# Autodesk Inventor assembly: LEG
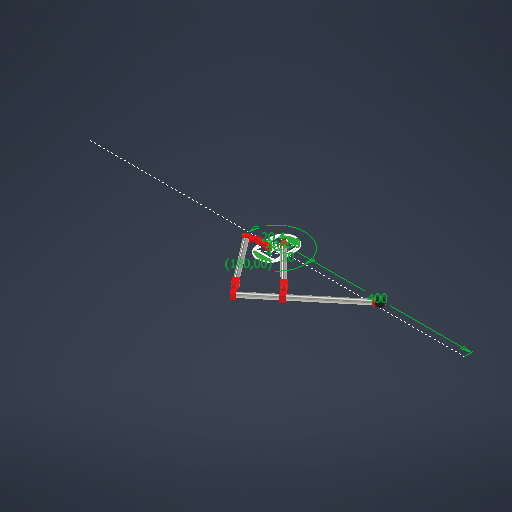
[picture p0: Inventor's stored thumbnail of the model, 512x512]
Saved by Autodesk Inventor 2027 (Build 310192060, 192F)
## iProperties
Created: 2026-08-01
Part Number: LEG
Document SubType Name: Assembly
Designer: User
Author: User
## Documents named in this file (11)
- G:\Github\Hot_dog\Hardware\Leg_concept\LEG.iam
- G:\Github\Hot_dog\Hardware\Leg_concept\Knee.ipt
- G:\Github\Hot_dog\Hardware\Leg_concept\foot.ipt
- G:\Github\Hot_dog\Hardware\Leg_concept\base.ipt
- G:\Github\Hot_dog\Hardware\Leg_concept\tibia.ipt
- G:\Github\Hot_dog\Hardware\Leg_concept\Connector_fill.ipt
- G:\Github\Hot_dog\Hardware\Leg_concept\Connector_hollow.ipt
- G:\Github\Hot_dog\Hardware\Leg_concept\short_tibia.ipt
- G:\Github\Hot_dog\Hardware\Leg_concept\connecting_rod.ipt
- G:\Github\Hot_dog\Hardware\Leg_concept\long_tibia.ipt
- G:\Github\Hot_dog\Hardware\Leg_concept\connector.ipt
## Components (14 placed, 10 different names)
1. Connector_fill:1 — Obrotowe:13, Obrotowe:29
2. Connector_hollow:1 — Obrotowe:23, Obrotowe:28
3. base:1 — Obrotowe:24, Obrotowe:25
4. Connector_hollow:2 — Obrotowe:15
5. tibia:2 — Obrotowe:26
6. connecting_rod:1 — Obrotowe:19, Obrotowe:24
7. connecting_rod:2 — Obrotowe:13, Obrotowe:25
8. Knee:1 — Obrotowe:21, Obrotowe:23
9. foot:1 — Obrotowe:18
10. Knee:2 — Obrotowe:15, Obrotowe:22
11. long_tibia:1 — Obrotowe:18, Obrotowe:21, Obrotowe:22
12. connector:1 — Obrotowe:19, Obrotowe:27
13. Knee:3 — Obrotowe:26, Obrotowe:27
14. short_tibia:1 — Obrotowe:28, Obrotowe:29
## Relationships (14: RevoluteJoint 13, WeldJoint 1)
- [WeldJoint]: Connector_hollow:2 ↔ tibia:2
- Obrotowe:13 [RevoluteJoint]: Connector_fill:1 ↔ connecting_rod:2
- Obrotowe:15 [RevoluteJoint]: Connector_hollow:2 ↔ Knee:2
- Obrotowe:18 [RevoluteJoint]: foot:1 ↔ long_tibia:1
- Obrotowe:19 [RevoluteJoint] (2 mm): connecting_rod:1 ↔ connector:1
- Obrotowe:21 [RevoluteJoint]: Knee:1 ↔ long_tibia:1
- Obrotowe:22 [RevoluteJoint]: Knee:2 ↔ long_tibia:1
- Obrotowe:23 [RevoluteJoint]: Connector_hollow:1 ↔ Knee:1
- Obrotowe:24 [RevoluteJoint]: base:1 ↔ connecting_rod:1
- Obrotowe:25 [RevoluteJoint]: base:1 ↔ connecting_rod:2
- Obrotowe:26 [RevoluteJoint]: tibia:2 ↔ Knee:3
- Obrotowe:27 [RevoluteJoint]: connector:1 ↔ Knee:3
- Obrotowe:28 [RevoluteJoint]: Connector_hollow:1 ↔ short_tibia:1
- Obrotowe:29 [RevoluteJoint]: Connector_fill:1 ↔ short_tibia:1
## Named parameters: d37_d35 = 0 mm
